# Autodesk Inventor assembly: Right_Arm
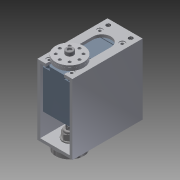
[picture p0: Inventor's stored thumbnail of the model, 180x180]
Saved by Autodesk Inventor 2013 (Build 170138000, 138)
## iProperties
Created: 2014-05-07
Part Number: Right_Arm
Document SubType Name: Assembly
Designer: andou
Author: andou
## Documents named in this file (10)
- C:\Users\andou\Documents\Inventor\RoboticsProject\project_4\Robot\Arm\Right_Arm.iam
- C:\Users\andou\Documents\Inventor\RoboticsProject\project_4\Robot\All Common\Serial_Case.ipt
- C:\Users\andou\Documents\Inventor\RoboticsProject\project_4\Robot\Arm\KRS-2542HV.ipt
- C:\Users\andou\Documents\Inventor\RoboticsProject\project_4\Robot\Arm\Horn_Spacer.ipt
- C:\Users\andou\Documents\Inventor\RoboticsProject\project_4\Robot\All Common\Cap(M3-6).ipt
- C:\Users\andou\Documents\Inventor\RoboticsProject\project_4\Robot\All Common\Cap(M4-15).ipt
- C:\Users\andou\Documents\Inventor\RoboticsProject\project_4\Robot\All Common\Nylon_Nat(M4).ipt
- C:\Users\andou\Documents\Inventor\RoboticsProject\project_4\Robot\All Common\Washer(M4).ipt
- C:\Users\andou\Documents\Inventor\RoboticsProject\project_4\Robot\Free_Horn\Free_Horn.iam
- C:\Users\andou\Documents\Inventor\RoboticsProject\project_4\Robot\All Common\Low_Height_Horn.ipt
## Components (9 placed, 9 different names)
1. Serial_Case:1 — 挿入:1, 挿入:2, 挿入:3, 挿入:5
2. KRS-2542HV:1 — 挿入:1, 挿入:2, 挿入:7
3. Horn_Spacer:1 — 挿入:8, 挿入:9, 挿入:10
4. Cap(M3-6):1 — 挿入:9
5. Cap(M4-15):1 — 挿入:6
6. Nylon_Nat(M4):1 — 挿入:4
7. Washer(M4):1 — 挿入:3, 挿入:4
8. Free_Horn:1 [sub-assembly] — 挿入:5, 挿入:6
9. Low_Height_Horn:1 — 挿入:7, 挿入:8, 挿入:10
## Relationships (10: Insert 10)
- 挿入:1 [Insert]: Serial_Case:1 ↔ KRS-2542HV:1
- 挿入:2 [Insert]: Serial_Case:1 ↔ KRS-2542HV:1
- 挿入:3 [Insert]: Serial_Case:1 ↔ Washer(M4):1
- 挿入:4 [Insert]: Nylon_Nat(M4):1 ↔ Washer(M4):1
- 挿入:5 [Insert]: Serial_Case:1 ↔ Free_Horn:1
- 挿入:6 [Insert]: Cap(M4-15):1 ↔ Free_Horn:1
- 挿入:7 [Insert]: KRS-2542HV:1 ↔ Low_Height_Horn:1
- 挿入:8 [Insert]: Horn_Spacer:1 ↔ Low_Height_Horn:1
- 挿入:9 [Insert]: Horn_Spacer:1 ↔ Cap(M3-6):1
- 挿入:10 [Insert]: Horn_Spacer:1 ↔ Low_Height_Horn:1
